# Autodesk Inventor assembly: EnsamblajeBarco
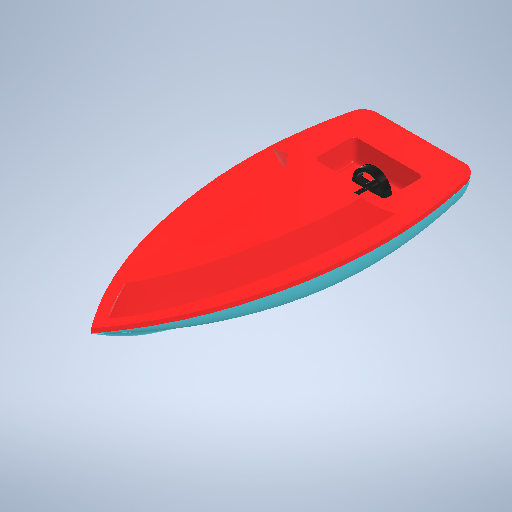
[picture p0: Inventor's stored thumbnail of the model, 512x512]
Saved by Autodesk Inventor 2025.2 (Build 292293000, 293)
## iProperties
Created: 2025-01-21
Part Number: EnsamblajeBarco
Document SubType Name: Assembly
Designer: usuario
Author: usuario
## Documents named in this file (5)
- C:\Users\usuario\Desktop\ModeladosAPM\BARCO\EnsamblajeBarco.iam
- C:\Users\usuario\Desktop\ModeladosAPM\BARCO\PiezabarcoInferior.ipt
- C:\Users\usuario\Desktop\ModeladosAPM\BARCO\Piezabarcosuperior.ipt
- C:\Users\usuario\Desktop\ModeladosAPM\BARCO\PiezaEjeTimon.ipt
- C:\Users\usuario\Desktop\ModeladosAPM\BARCO\PiezaTimon.ipt
## Components (4 placed, 4 different names)
1. PiezabarcoInferior:1 — Coincidencia:1, Coincidencia:2, Coincidencia:3
2. Piezabarcosuperior:1 — Coincidencia:1, Coincidencia:2, Coincidencia:3, Coincidencia:4, Coincidencia:5, Coincidencia:6
3. PiezaEjeTimon:1 — Coincidencia:4, Coincidencia:5, Coincidencia:6, Coincidencia:7
4. PiezaTimon:1 — Coincidencia:7
## Relationships (7: Mate 7)
- Coincidencia:1 [Mate]: PiezabarcoInferior:1 ↔ Piezabarcosuperior:1
- Coincidencia:2 [Mate]: PiezabarcoInferior:1 ↔ Piezabarcosuperior:1
- Coincidencia:3 [Mate]: PiezabarcoInferior:1 ↔ Piezabarcosuperior:1
- Coincidencia:4 [Mate]: Piezabarcosuperior:1 ↔ PiezaEjeTimon:1
- Coincidencia:5 [Mate]: Piezabarcosuperior:1 ↔ PiezaEjeTimon:1
- Coincidencia:6 [Mate]: Piezabarcosuperior:1 ↔ PiezaEjeTimon:1
- Coincidencia:7 [Mate]: PiezaEjeTimon:1 ↔ PiezaTimon:1
